# Autodesk Inventor assembly: RearGearboxAssembly_MIR
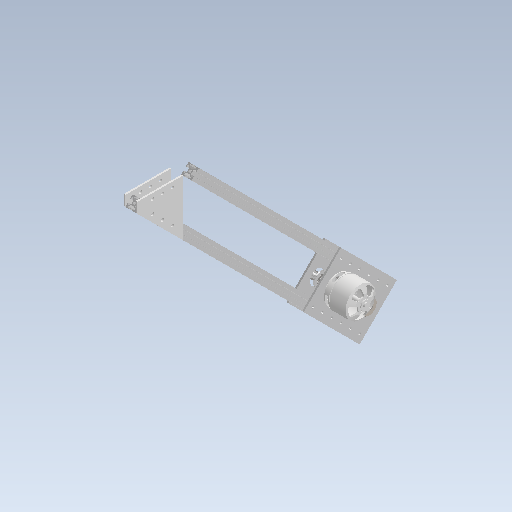
[picture p0: Inventor's stored thumbnail of the model, 512x512]
Saved by Autodesk Inventor 2023 (Build 270158000, 158)
## iProperties
Created: 2023-02-14
Part Number: RearGearboxAssembly_MIR
Document SubType Name: Assembly
Designer: Dave
Author: Dave
## Documents named in this file (6)
- C:\Users\Dave\Documents\GitHub\BehrendURCMechanical\CAD\Chassis\GearBox\Final Gears and Assemblies\RearGearboxAssembly_MIR.iam
- C:\Users\Dave\Documents\GitHub\BehrendURCMechanical\CAD\Chassis\GearBox\Final Gears and Assemblies\Gearbox Assembly_MIR.iam
- C:\Users\Dave\Documents\GitHub\BehrendURCMechanical\CAD\Chassis\CH-1-01-FrontKneeJoint_MIR.ipt
- C:\Users\Dave\Documents\GitHub\BehrendURCMechanical\CAD\Chassis\CH-1-01-20x20 Channel\CH-1-01-20x20 Channel-604.ipt
- C:\Users\Dave\Documents\GitHub\BehrendURCMechanical\CAD\Chassis\CH-1-01-20x20 Channel.ipt
- C:\Users\Dave\Documents\GitHub\BehrendURCMechanical\CAD\Chassis\CH-1-01-20x20 Channel\CH-1-01-20x20 Channel-528.ipt
## Components (5 placed, 4 different names)
1. Gearbox Assembly_MIR:1 [sub-assembly] — Angle:1, Flush:10, Mate:1, Flush:9, Flush:14, Flush:13, Mate:5, Flush:12
2. CH-1-01-FrontKneeJoint_MIR:1 — Flush:8, Flush:7, Mate:3, Flush:11
3. CH-1-01-FrontKneeJoint_MIR:2 — Flush:8, Flush:7, Mate:4, Mate:2
4. CH-1-01-20x20 Channel-604:1 — Mate:4, Mate:3, Mate:2, Flush:11, Flush:10, Mate:1, Flush:9
5. CH-1-01-20x20 Channel-528:2 — Flush:14, Flush:13, Mate:5, Flush:12
## Relationships (14: Flush 8, Mate 5, Angle 1)
- Angle:1 (45 deg): Gearbox Assembly_MIR:1
- Flush:8: CH-1-01-FrontKneeJoint_MIR:1 ↔ CH-1-01-FrontKneeJoint_MIR:2
- Flush:7: CH-1-01-FrontKneeJoint_MIR:1 ↔ CH-1-01-FrontKneeJoint_MIR:2
- Mate:4: CH-1-01-FrontKneeJoint_MIR:2 ↔ CH-1-01-20x20 Channel-604:1
- Mate:3: CH-1-01-FrontKneeJoint_MIR:1 ↔ CH-1-01-20x20 Channel-604:1
- Mate:2: CH-1-01-FrontKneeJoint_MIR:2 ↔ CH-1-01-20x20 Channel-604:1
- Flush:11: CH-1-01-FrontKneeJoint_MIR:1 ↔ CH-1-01-20x20 Channel-604:1
- Flush:10 (2.6924 mm): Gearbox Assembly_MIR:1 ↔ CH-1-01-20x20 Channel-604:1
- Mate:1 (3.3 mm): Gearbox Assembly_MIR:1 ↔ CH-1-01-20x20 Channel-604:1
- Flush:9: Gearbox Assembly_MIR:1 ↔ CH-1-01-20x20 Channel-604:1
- Flush:14: Gearbox Assembly_MIR:1 ↔ CH-1-01-20x20 Channel-528:2
- Flush:13 (2.6924 mm): Gearbox Assembly_MIR:1 ↔ CH-1-01-20x20 Channel-528:2
- Mate:5 (3.3 mm): Gearbox Assembly_MIR:1 ↔ CH-1-01-20x20 Channel-528:2
- Flush:12: Gearbox Assembly_MIR:1 ↔ CH-1-01-20x20 Channel-528:2
